# Autodesk Inventor assembly: ASY NVPH-320 joint flange
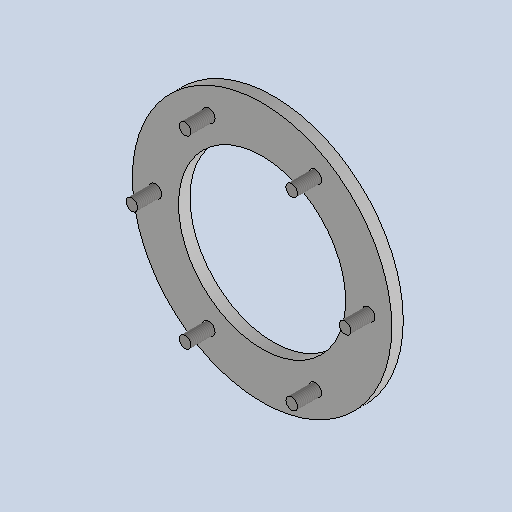
[picture p0: Inventor's stored thumbnail of the model, 512x512]
Saved by Autodesk Inventor 2025 (Build 290162010, 162A)
## iProperties
Created: 2024-12-03
Part Number: ASY NVPH-320 joint flange
Document SubType Name: Assembly
Designer: admin
Author: admin
## Documents named in this file (4)
- C:\Users\admin\YandexDisk-badmisterfox\домашниий пк\Inventor\NDM-VOS_powder_hopper\ASY NVPH-466 joint flange.iam
- C:\Users\admin\YandexDisk-badmisterfox\домашниий пк\Inventor\NDM-VOS_powder_hopper\NVPH-413 revision steel circle.ipt
- C:\Users\admin\YandexDisk-badmisterfox\домашниий пк\Inventor\NDM-VOS_powder_hopper\NVPH-412 revision plastic circle.ipt
- C:\Users\admin\YandexDisk-badmisterfox\домашниий пк\Inventor\Content Center Files\en-US\DIN 976-1 A\DIN 976-1 - M10 x 30 - A.ipt
## Components (8 placed, 3 different names)
1. ДМФ 041 кольцо под шпильки КОРМА:1 — Mate:1, Mate:2, Flush:1, Rigid:1
2. ДМФ 025 кольцо прижимное корма наружное:1 — Rigid:1
3. DIN 976-1 - M10 x 30 - A:1
4. DIN 976-1 - M10 x 30 - A:2
5. DIN 976-1 - M10 x 30 - A:3
6. DIN 976-1 - M10 x 30 - A:4
7. DIN 976-1 - M10 x 30 - A:5
8. DIN 976-1 - M10 x 30 - A:6
## Relationships (10: RevoluteJoint 6, Mate 2, Flush 1, WeldJoint 1)
- [RevoluteJoint]: ДМФ 041 кольцо под шпильки КОРМА:1 ↔ DIN 976-1 - M10 x 30 - A:1
- [RevoluteJoint]: ДМФ 041 кольцо под шпильки КОРМА:1 ↔ DIN 976-1 - M10 x 30 - A:2
- [RevoluteJoint]: ДМФ 041 кольцо под шпильки КОРМА:1 ↔ DIN 976-1 - M10 x 30 - A:3
- [RevoluteJoint]: ДМФ 041 кольцо под шпильки КОРМА:1 ↔ DIN 976-1 - M10 x 30 - A:6
- [RevoluteJoint]: ДМФ 041 кольцо под шпильки КОРМА:1 ↔ DIN 976-1 - M10 x 30 - A:4
- [RevoluteJoint]: ДМФ 041 кольцо под шпильки КОРМА:1 ↔ DIN 976-1 - M10 x 30 - A:5
- Mate:1: ДМФ 041 кольцо под шпильки КОРМА:1
- Mate:2: ДМФ 041 кольцо под шпильки КОРМА:1
- Flush:1: ДМФ 041 кольцо под шпильки КОРМА:1
- Rigid:1 [WeldJoint]: ДМФ 041 кольцо под шпильки КОРМА:1 ↔ ДМФ 025 кольцо прижимное корма наружное:1
